# Autodesk Inventor assembly: assembly
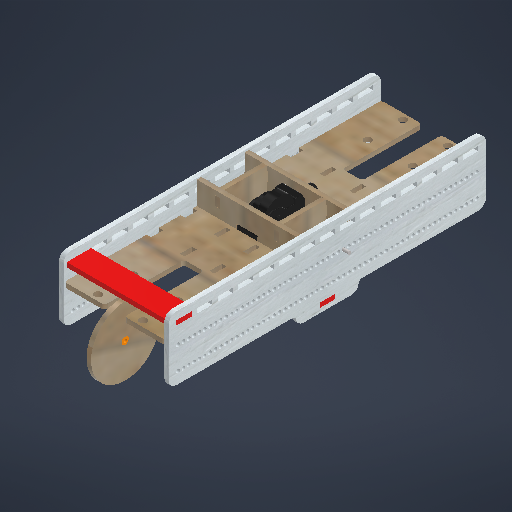
[picture p0: Inventor's stored thumbnail of the model, 512x512]
Saved by Autodesk Inventor 2025.3 (Build 293356030, 356C)
## iProperties
Created: 2025-10-01
Part Number: assembly
Document SubType Name: Assembly
Designer: 陳泓任
Author: 陳泓任
## Documents named in this file (10)
- C:\Users\Ou918\3D-model-temp\introduction to mechanical engineering(1)\version_5\assembly.iam
- C:\Users\Ou918\3D-model-temp\introduction to mechanical engineering(1)\version_5\main_frame.ipt
- C:\Users\Ou918\3D-model-temp\introduction to mechanical engineering(1)\version_5\baffle_back.ipt
- C:\Users\Ou918\3D-model-temp\introduction to mechanical engineering(1)\version_5\baffle_front.ipt
- C:\Users\Ou918\3D-model-temp\introduction to mechanical engineering(1)\version_5\support_edited.ipt
- C:\Users\Ou918\3D-model-temp\introduction to mechanical engineering(1)\version_5\bolt.ipt
- C:\Users\Ou918\3D-model-temp\introduction to mechanical engineering(1)\version_5\side_frame.ipt
- C:\Users\Ou918\3D-model-temp\introduction to mechanical engineering(1)\發條組合\發條組合.iam
- C:\Users\Ou918\3D-model-temp\introduction to mechanical engineering(1)\version_5\beam.ipt
- C:\Users\Ou918\3D-model-temp\introduction to mechanical engineering(1)\45mm wheel(with sleeve).iam
## Components (12 placed, 9 different names)
1. main_frame:1 — 貼合:1, 貼合:2, 貼合:3, 貼合:4, 貼合:5, 貼合:6, 貼合:7, 貼合:10, 貼合:11, 貼合:17, 貼合:18, 貼合:19, 貼合:22, 貼合:24, 貼合:31
2. 發條組合:1 [sub-assembly] — 貼合:18, 貼合:19, 貼合:20, 貼合:27
3. side_frame:1 — 齊平:1, 貼合:24, 齊平:2, 貼合:25, 齊平:3, 貼合:26, 貼合:27, 貼合:28, 齊平:4, 貼合:29, 貼合:30
4. side_frame:2 — 齊平:1, 貼合:22, 齊平:2
5. baffle_back:1 — 貼合:1, 貼合:2, 貼合:3
6. baffle_front:1 — 貼合:4, 貼合:5, 貼合:6, 貼合:8, 貼合:16, 貼合:20
7. support_edited:1 — 貼合:7, 貼合:8, 貼合:13, 貼合:14, 貼合:16
8. support_edited:2 — 貼合:10, 貼合:11, 貼合:15, 貼合:17
9. bolt:1 — 貼合:13, 貼合:14, 貼合:15
10. beam:1 — 貼合:25, 齊平:3, 貼合:26
11. 45mm wheel(with sleeve):1 [sub-assembly] — 貼合:28, 貼合:31
12. beam:2 — 齊平:4, 貼合:29, 貼合:30
## Relationships (31: Mate 27, Flush 4)
- 貼合:1 [Mate]: main_frame:1 ↔ baffle_back:1
- 貼合:2 [Mate]: main_frame:1 ↔ baffle_back:1
- 貼合:3 [Mate]: main_frame:1 ↔ baffle_back:1
- 貼合:4 [Mate]: main_frame:1 ↔ baffle_front:1
- 貼合:5 [Mate]: main_frame:1 ↔ baffle_front:1
- 貼合:6 [Mate]: main_frame:1 ↔ baffle_front:1
- 貼合:7 [Mate]: main_frame:1 ↔ support_edited:1
- 貼合:8 [Mate]: baffle_front:1 ↔ support_edited:1
- 貼合:10 [Mate]: main_frame:1 ↔ support_edited:2
- 貼合:11 [Mate]: main_frame:1 ↔ support_edited:2
- 貼合:13 [Mate]: support_edited:1 ↔ bolt:1
- 貼合:14 [Mate]: support_edited:1 ↔ bolt:1
- 貼合:15 [Mate]: support_edited:2 ↔ bolt:1
- 貼合:16 [Mate]: baffle_front:1 ↔ support_edited:1
- 貼合:17 [Mate]: main_frame:1 ↔ support_edited:2
- 貼合:18 [Mate]: main_frame:1 ↔ 發條組合:1
- 貼合:19 [Mate]: main_frame:1 ↔ 發條組合:1
- 貼合:20 [Mate]: 發條組合:1 ↔ baffle_front:1
- 齊平:1 [Flush]: side_frame:1 ↔ side_frame:2
- 貼合:22 [Mate]: main_frame:1 ↔ side_frame:2
- 貼合:24 [Mate]: main_frame:1 ↔ side_frame:1
- 齊平:2 [Flush]: side_frame:1 ↔ side_frame:2
- 貼合:25 [Mate]: side_frame:1 ↔ beam:1
- 齊平:3 [Flush]: side_frame:1 ↔ beam:1
- 貼合:26 [Mate]: side_frame:1 ↔ beam:1
- 貼合:27 [Mate]: 發條組合:1 ↔ side_frame:1
- 貼合:28 [Mate]: side_frame:1 ↔ 45mm wheel(with sleeve):1
- 齊平:4 [Flush]: side_frame:1 ↔ beam:2
- 貼合:29 [Mate]: side_frame:1 ↔ beam:2
- 貼合:30 [Mate]: side_frame:1 ↔ beam:2
- 貼合:31 [Mate]: main_frame:1 ↔ 45mm wheel(with sleeve):1
